# Autodesk Inventor assembly: Gesamtzusammensetzung
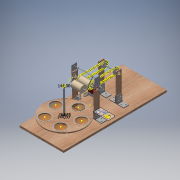
[picture p0: Inventor's stored thumbnail of the model, 180x180]
Saved by Autodesk Inventor 2018 (Build 220112000, 112)
## iProperties
Created: 2018-03-14
Part Number: Gesamtzusammensetzung
Material: Generisch
Document SubType Name: Assembly
Designer: Julian
Author: Julian
## Documents named in this file (6)
- C:\Users\Dominik\Desktop\Diplomarbeit\fuettr_prototype\Mechanical\Inventorskizzen\Gesamtzusammensetzung.iam
- C:\Users\Dominik\Desktop\Diplomarbeit\fuettr_prototype\Mechanical\Inventorskizzen\Grundplatte.ipt
- C:\Users\Dominik\Desktop\Diplomarbeit\fuettr_prototype\Mechanical\Inventorskizzen\Plattenzusammensetzung.iam
- C:\Users\Dominik\Desktop\Diplomarbeit\fuettr_prototype\Mechanical\Inventorskizzen\Förderband.iam
- C:\Users\Dominik\Desktop\Diplomarbeit\fuettr_prototype\Mechanical\Inventorskizzen\Draht.ipt
- C:\Users\Dominik\Desktop\Diplomarbeit\fuettr_prototype\Mechanical\Inventorskizzen\Draht_Halterung.ipt
## Components (6 placed, 5 different names)
1. Grundplatte:2 — Drehbar:1, Drehbar:2, Passend:1, Passend:3, Passend:4, Passend:5, Passend:7, Passend:8, Passend:10, Passend:11
2. Plattenzusammensetzung:1 [sub-assembly] — Drehbar:1
3. Förderband:1 [sub-assembly] — Drehbar:2
4. Draht:1 — Passend:1, Passend:2, Passend:6, Passend:9
5. Draht_Halterung:1 — Passend:2, Passend:3, Passend:4, Passend:5, Passend:6
6. Draht_Halterung:2 — Passend:7, Passend:8, Passend:9, Passend:10, Passend:11
## Relationships (13: Mate 11, RevoluteJoint 2)
- Drehbar:1 [RevoluteJoint]: Grundplatte:2 ↔ Plattenzusammensetzung:1
- Drehbar:2 [RevoluteJoint]: Grundplatte:2 ↔ Förderband:1
- Passend:1 [Mate]: Grundplatte:2 ↔ Draht:1
- Passend:2 [Mate]: Draht:1 ↔ Draht_Halterung:1
- Passend:3 [Mate]: Grundplatte:2 ↔ Draht_Halterung:1
- Passend:4 [Mate]: Grundplatte:2 ↔ Draht_Halterung:1
- Passend:5 [Mate]: Grundplatte:2 ↔ Draht_Halterung:1
- Passend:6 [Mate]: Draht:1 ↔ Draht_Halterung:1
- Passend:7 [Mate]: Grundplatte:2 ↔ Draht_Halterung:2
- Passend:8 [Mate]: Grundplatte:2 ↔ Draht_Halterung:2
- Passend:9 [Mate]: Draht:1 ↔ Draht_Halterung:2
- Passend:10 [Mate]: Grundplatte:2 ↔ Draht_Halterung:2
- Passend:11 [Mate]: Grundplatte:2 ↔ Draht_Halterung:2
